# Autodesk Inventor assembly: Axel Assembly
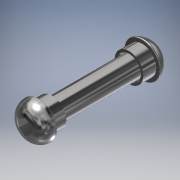
[picture p0: Inventor's stored thumbnail of the model, 180x180]
Saved by Autodesk Inventor 2018 (Build 220112000, 112)
## iProperties
Created: 2018-03-01
Part Number: Axel Assembly
Document SubType Name: Assembly
Designer: 232963
Author: 232963
## Documents named in this file (4)
- P:\IED\SchoolCAD\ReverseEngineering\Axel Assembly.iam
- P:\IED\SchoolCAD\ReverseEngineering\Axel Buffer.ipt
- P:\IED\SchoolCAD\ReverseEngineering\Axel-Male.ipt
- P:\IED\SchoolCAD\ReverseEngineering\Axel-Female.ipt
## Components (4 placed, 3 different names)
1. Axel Buffer:1 — Insert:1
2. Axel Buffer:2 — Insert:3
3. Axel-Male:1 — Insert:1, Insert:2
4. Axel-Female:1 — Insert:2, Insert:3
## Relationships (3: Insert 3)
- Insert:1: Axel Buffer:1 ↔ Axel-Male:1
- Insert:2: Axel-Male:1 ↔ Axel-Female:1
- Insert:3: Axel Buffer:2 ↔ Axel-Female:1
